# Autodesk Inventor assembly: Scrambler II
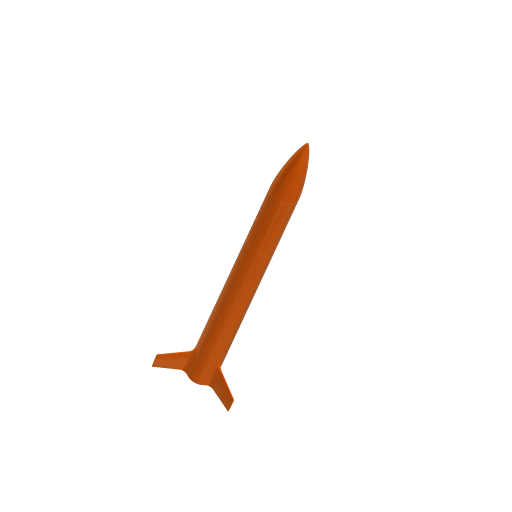
[picture p0: Inventor's stored thumbnail of the model, 512x512]
Saved by Autodesk Inventor 2024 (Build 280153000, 153)
## iProperties
Created: 2023-12-30
Part Number: Scrambler II
Document SubType Name: Assembly
Designer: Jamie
Mass: 631.455 g
Surface Area: 5625.65 cm^2
Volume: 391.502 cm^3
Density: 1.6129 g/cm^3
Author: Jamie
## Documents named in this file (6)
- C:\Users\Jamie\Documents\Uni\DARE\Scrambler-2-CAD\Hide and seek\Dummy Scrambler.iam
- C:\Users\Jamie\Documents\Uni\DARE\Scrambler-2-CAD\Hide and seek\Lower skin.ipt
- C:\Users\Jamie\Documents\Uni\DARE\Scrambler-2-CAD\Hide and seek\Upper skin.ipt
- C:\Users\Jamie\Documents\Uni\DARE\Scrambler-2-CAD\Hide and seek\Nosecone.ipt
- C:\Users\Jamie\Documents\Uni\DARE\Scrambler-2-CAD\Hide and seek\Engine skin glued.iam
- Engine skin.iam
## Components (4 placed, 4 different names)
1. Lower skin:1 — Mate:1, Mate:2, Mate:3, Mate:4, Mate:5, Mate:6
2. Upper skin:1 — Mate:1, Mate:2, Mate:3, Mate:7, Mate:8, Mate:9
3. Nosecone:1 — Mate:7, Mate:8, Mate:9
4. Engine skin:1 [sub-assembly] — Mate:4, Mate:5, Mate:6
## Relationships (9: Mate 9)
- Mate:1: Lower skin:1 ↔ Upper skin:1
- Mate:2: Lower skin:1 ↔ Upper skin:1
- Mate:3: Lower skin:1 ↔ Upper skin:1
- Mate:4: Lower skin:1 ↔ Engine skin:1
- Mate:5: Lower skin:1 ↔ Engine skin:1
- Mate:6: Lower skin:1 ↔ Engine skin:1
- Mate:7: Upper skin:1 ↔ Nosecone:1
- Mate:8: Upper skin:1 ↔ Nosecone:1
- Mate:9: Upper skin:1 ↔ Nosecone:1
